# Autodesk Inventor assembly: RPIassem
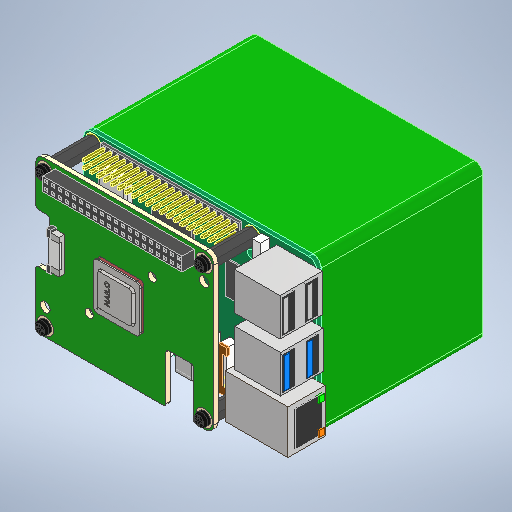
[picture p0: Inventor's stored thumbnail of the model, 512x512]
Saved by Autodesk Inventor 2025.1 (Build 291241000, 241)
## iProperties
Created: 2025-05-22
Part Number: RPIassem
Document SubType Name: Assembly
Designer: User
Author: User
## Documents named in this file (4)
- D:\One Drive\OneDrive - Politeknik Sultan Salahuddin Abdul Aziz Shah\Documents\Inventor\RobosotPSA\RPIassem.iam
- D:\One Drive\OneDrive - Politeknik Sultan Salahuddin Abdul Aziz Shah\Documents\Inventor\RobosotPSA\raspberry-pi-5-sbc-simple\raspberry-pi-5-sbc-simple\raspberry-pi-5-sbc-simple.ipt
- D:\One Drive\OneDrive - Politeknik Sultan Salahuddin Abdul Aziz Shah\Documents\Inventor\RobosotPSA\RPiAIHATPlus\RPiAIHATPlus\RPiAIHATPlus.ipt
- D:\One Drive\OneDrive - Politeknik Sultan Salahuddin Abdul Aziz Shah\Documents\Inventor\RobosotPSA\UPSboard.ipt
## Components (3 placed, 3 different names)
1. raspberry-pi-5-sbc-simple:1 — Mate:1, Mate:2, Mate:3, Flush:1
2. RPiAIHATPlus:1 — Mate:1, Mate:2, Mate:3
3. UPSboard:1 — Flush:1
## Relationships (4: Mate 3, Flush 1)
- Mate:1: raspberry-pi-5-sbc-simple:1 ↔ RPiAIHATPlus:1
- Mate:2: raspberry-pi-5-sbc-simple:1 ↔ RPiAIHATPlus:1
- Mate:3: raspberry-pi-5-sbc-simple:1 ↔ RPiAIHATPlus:1
- Flush:1: raspberry-pi-5-sbc-simple:1 ↔ UPSboard:1
